# Autodesk Inventor assembly: pullBoxPower
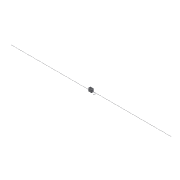
[picture p0: Inventor's stored thumbnail of the model, 180x180]
Saved by Autodesk Inventor 2016 (Build 200138000, 138)
## iProperties
Created: 2014-12-12
Part Number: pullBoxPower
Document SubType Name: Assembly
Designer: Dave
Author: Dave
## Documents named in this file (7)
- C:\Users\krosie\Google Drive\HERA\hera-cad\Node\pullBoxPower.iam
- C:\Users\krosie\Google Drive\HERA\hera-cad\Node\pullboxPower.ipt
- C:\Users\krosie\Google Drive\HERA\hera-cad\Node\pipe_50mm_0.5m.ipt
- C:\Users\krosie\Google Drive\HERA\hera-cad\Node\pipe_50mm_1.5m.ipt
- C:\Users\krosie\Google Drive\HERA\hera-cad\Node\sweep_50mm.ipt
- C:\Users\krosie\Google Drive\HERA\hera-cad\Node\pullboxPowerLid.ipt
- C:\Users\krosie\Google Drive\HERA\hera-cad\Node\pipe_50mm_Long.ipt
## Components (10 placed, 6 different names)
1. pullboxPower:2 — Insert:1, Insert:2, Insert:3, Angle:1, Angle:2, Flush:1, Flush:2, Mate:1
2. pipe_50mm_0.5m:1 — Insert:3, Insert:4
3. pipe_50mm_1.5m:1 — Insert:1, Insert:9
4. pipe_50mm_1.5m:2 — Insert:2, Insert:10
5. sweep_50mm:1 — Insert:4, Angle:1, Insert:8
6. sweep_50mm:2 — Angle:2, Insert:7, Insert:8
7. pipe_50mm_0.5m:3 — Insert:7
8. pullboxPowerLid:1 — Flush:1, Flush:2, Mate:1
9. pipe_50mm_Long:1 — Insert:10
10. pipe_50mm_Long:2 — Insert:9
## Relationships (13: Insert 8, Angle 2, Flush 2, Mate 1)
- Insert:1: pullboxPower:2 ↔ pipe_50mm_1.5m:1
- Insert:2: pullboxPower:2 ↔ pipe_50mm_1.5m:2
- Insert:3: pullboxPower:2 ↔ pipe_50mm_0.5m:1
- Insert:4: pipe_50mm_0.5m:1 ↔ sweep_50mm:1
- Angle:1 (0 deg): pullboxPower:2 ↔ sweep_50mm:1
- Angle:2 (180 deg): pullboxPower:2 ↔ sweep_50mm:2
- Insert:7 (-101.6 mm): sweep_50mm:2 ↔ pipe_50mm_0.5m:3
- Flush:1: pullboxPower:2 ↔ pullboxPowerLid:1
- Flush:2: pullboxPower:2 ↔ pullboxPowerLid:1
- Mate:1 (5.08 mm): pullboxPower:2 ↔ pullboxPowerLid:1
- Insert:8 (-101.6 mm): sweep_50mm:1 ↔ sweep_50mm:2
- Insert:9: pipe_50mm_1.5m:1 ↔ pipe_50mm_Long:2
- Insert:10: pipe_50mm_1.5m:2 ↔ pipe_50mm_Long:1
